# Autodesk Inventor assembly: Assembly_Opentrons_Microscope
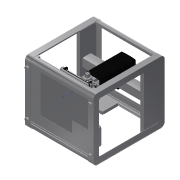
[picture p0: Inventor's stored thumbnail of the model, 180x180]
Saved by Autodesk Inventor 2019.4 (Build 234330000, 330)
## iProperties
Created: 2021-03-18
Part Number: Assembly_Opentrons_Microscope
Document SubType Name: Assembly
Designer: diederichbenedict
Author: diederichbenedict
## Documents named in this file (3)
- C:\Users\diederichbenedict\Dropbox\Dokumente\Promotion\PROJECTS\OPENTRONS\INVENTOR\Assembly_Opentrons_Microscope.iam
- C:\Users\diederichbenedict\Dropbox\Dokumente\Promotion\PROJECTS\OPENTRONS\INVENTOR\OT-2 Reference Model Detailed.ipt
- C:\Users\diederichbenedict\Dropbox\Dokumente\Promotion\PROJECTS\OPENTRONS\INVENTOR\Assembly_Opentrons_Imagingunit_v3.iam
## Components (2 placed, 2 different names)
1. OT-2 Reference Model Detailed:1 — Mate:1, Mate:2, Mate:3
2. Assembly_Opentrons_Imagingunit_v3:1 [sub-assembly] — Mate:1, Mate:2, Mate:3
## Relationships (3: Mate 3)
- Mate:1 (10 mm): OT-2 Reference Model Detailed:1 ↔ Assembly_Opentrons_Imagingunit_v3:1
- Mate:2: OT-2 Reference Model Detailed:1 ↔ Assembly_Opentrons_Imagingunit_v3:1
- Mate:3: OT-2 Reference Model Detailed:1 ↔ Assembly_Opentrons_Imagingunit_v3:1
